# Autodesk Inventor assembly: Clippers
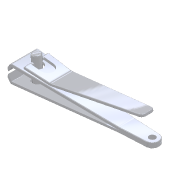
[picture p0: Inventor's stored thumbnail of the model, 180x180]
Saved by Autodesk Inventor 2020.1 (Build 241239000, 239)
## iProperties
Created: 2010-10-13
Part Number: Clippers
Document SubType Name: Assembly
Designer: Thom Tremblay
Author: Thom Tremblay
## Documents named in this file (5)
- C:\Users\thom_tremblay\Desktop\Inventor ACP Data\Clippers.iam
- C:\Users\thom_tremblay\Desktop\Inventor ACP Data\Parts\Constraint Plane.ipt
- C:\Users\thom_tremblay\Desktop\Inventor ACP Data\Parts\Clipper Blade.ipt
- C:\Users\thom_tremblay\Desktop\Inventor ACP Data\Parts\Pin.ipt
- C:\Users\thom_tremblay\Desktop\Inventor ACP Data\Parts\Lever.ipt
## Components (6 placed, 4 different names)
1. Constraint Plane:1 — Mate:1, Drive This Constraint, Mate:3, Flush:2
2. Constraint Plane:2 — Mate:1, Drive This Constraint, Mate:3, Flush:1
3. Clipper Blade:1 — Flush:1, Flush:2, Insert:1, Mate:4, Mate:5, Tangent:1
4. Clipper Blade:2 — Insert:1, Angle:1, Insert:2
5. Pin:1 — Insert:2, Mate:6, Mate:7
6. Lever:1 — Mate:6, Tangent:1, Mate:7
## Relationships (13: Mate 7, Flush 2, Insert 2, Angle 1, Tangent 1)
- Mate:1: Constraint Plane:1 ↔ Constraint Plane:2
- Drive This Constraint [Mate] (1.27 mm): Constraint Plane:1 ↔ Constraint Plane:2
- Mate:3: Constraint Plane:1 ↔ Constraint Plane:2
- Flush:1: Constraint Plane:2 ↔ Clipper Blade:1
- Flush:2: Constraint Plane:1 ↔ Clipper Blade:1
- Insert:1: Clipper Blade:1 ↔ Clipper Blade:2
- Angle:1 (180 deg): Clipper Blade:2
- Mate:4: Clipper Blade:1
- Mate:5: Clipper Blade:1
- Insert:2: Clipper Blade:2 ↔ Pin:1
- Mate:6: Pin:1 ↔ Lever:1
- Tangent:1: Clipper Blade:1 ↔ Lever:1
- Mate:7: Pin:1 ↔ Lever:1
